# Autodesk Inventor assembly: ENSAMBLE DEL MOLDE DE INYECCION
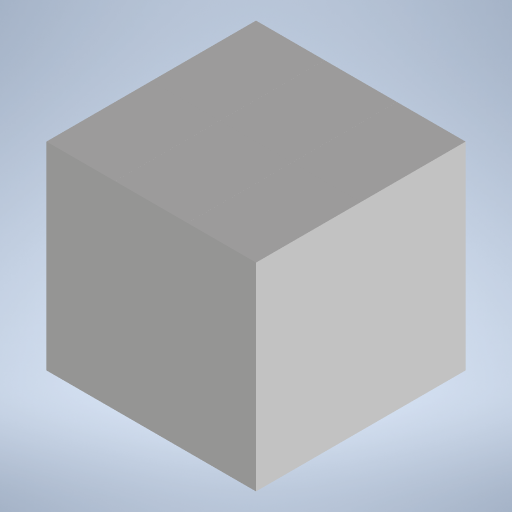
[picture p0: Inventor's stored thumbnail of the model, 512x512]
Saved by Autodesk Inventor 2024 (Build 280153000, 153)
## iProperties
Created: 2023-08-25
Part Number: ENSAMBLE DEL MOLDE DE INYECCION
Document SubType Name: Assembly
Designer: gdpg
Author: gdpg
## Documents named in this file (19)
- C:\Users\gdpg\Desktop\MANIQUI\MODELO FINAL\MOLDE\ENSAMBLE DEL MOLDE DE INYECCION.iam
- C:\Users\gdpg\Desktop\MANIQUI\MODELO FINAL\MOLDE\1.ipt
- C:\Users\gdpg\Desktop\MANIQUI\MODELO FINAL\MOLDE\2.ipt
- C:\Users\gdpg\Desktop\MANIQUI\MODELO FINAL\MOLDE\3.ipt
- C:\Users\gdpg\Desktop\MANIQUI\MODELO FINAL\MOLDE\4.ipt
- C:\Users\gdpg\Desktop\MANIQUI\MODELO FINAL\MOLDE\11.ipt
- C:\Users\gdpg\Desktop\MANIQUI\MODELO FINAL\MOLDE\12.ipt
- C:\Users\gdpg\Desktop\MANIQUI\MODELO FINAL\MOLDE\7.ipt
- C:\Users\gdpg\Desktop\MANIQUI\MODELO FINAL\MOLDE\8.ipt
- C:\Users\gdpg\Desktop\MANIQUI\MODELO FINAL\MOLDE\5.ipt
- C:\Users\gdpg\Desktop\MANIQUI\MODELO FINAL\MOLDE\6.ipt
- C:\Users\gdpg\Desktop\MANIQUI\MODELO FINAL\MOLDE\9.ipt
- C:\Users\gdpg\Desktop\MANIQUI\MODELO FINAL\MOLDE\10.ipt
- C:\Users\gdpg\Desktop\MANIQUI\MODELO FINAL\MOLDE\13.ipt
- C:\Users\gdpg\Desktop\MANIQUI\MODELO FINAL\MOLDE\14.ipt
- C:\Users\gdpg\Desktop\MANIQUI\MODELO FINAL\MOLDE\15.ipt
- C:\Users\gdpg\Desktop\MANIQUI\MODELO FINAL\MOLDE\16.ipt
- C:\Users\gdpg\Desktop\MANIQUI\MODELO FINAL\MOLDE\17.ipt
- C:\Users\gdpg\Desktop\MANIQUI\MODELO FINAL\MOLDE\18.ipt
## Components (18 placed, 18 different names)
1. 1:1 — Nivelación:1, Coincidencia:1, Coincidencia:2, Coincidencia:15, Coincidencia:16, Coincidencia:19, Coincidencia:20, Coincidencia:23, Coincidencia:28, Coincidencia:32
2. 2:1 — Nivelación:1, Coincidencia:5, Coincidencia:6, Coincidencia:26, Coincidencia:29
3. 3:1 — Coincidencia:19, Coincidencia:20, Coincidencia:21, Coincidencia:22, Coincidencia:31
4. 4:1 — Coincidencia:21, Coincidencia:22, Coincidencia:33
5. 5:1 — Coincidencia:13, Coincidencia:14, Coincidencia:24
6. 6:1 — Coincidencia:11, Coincidencia:12
7. 7:1 — Coincidencia:1, Coincidencia:2, Coincidencia:3, Coincidencia:4, Coincidencia:7, Coincidencia:8, Coincidencia:13, Coincidencia:14
8. 8:1 — Coincidencia:3, Coincidencia:4, Coincidencia:5, Coincidencia:6, Coincidencia:11, Coincidencia:12
9. 9:1 — Coincidencia:15, Coincidencia:16, Coincidencia:17, Coincidencia:18
10. 10:1 — Coincidencia:17, Coincidencia:18
11. 11:1 — Coincidencia:7, Coincidencia:8, Coincidencia:9, Coincidencia:10, Coincidencia:27
12. 12:1 — Coincidencia:9, Coincidencia:10, Coincidencia:30
13. 13:1 — Coincidencia:23, Coincidencia:24, Coincidencia:25
14. 14:1 — Coincidencia:25, Coincidencia:26
15. 15:1 — Coincidencia:27, Coincidencia:28
16. 16:1 — Coincidencia:29, Coincidencia:30
17. 17:1 — Coincidencia:31, Coincidencia:32, Coincidencia:34
18. 18:1 — Coincidencia:33, Coincidencia:34
## Relationships (35: Mate 34, Flush 1)
- Nivelación:1 [Flush]: 1:1 ↔ 2:1
- Coincidencia:1 [Mate]: 1:1 ↔ 7:1
- Coincidencia:2 [Mate]: 1:1 ↔ 7:1
- Coincidencia:3 [Mate]: 7:1 ↔ 8:1
- Coincidencia:4 [Mate]: 7:1 ↔ 8:1
- Coincidencia:5 [Mate]: 2:1 ↔ 8:1
- Coincidencia:6 [Mate]: 2:1 ↔ 8:1
- Coincidencia:7 [Mate]: 7:1 ↔ 11:1
- Coincidencia:8 [Mate]: 7:1 ↔ 11:1
- Coincidencia:9 [Mate]: 11:1 ↔ 12:1
- Coincidencia:10 [Mate]: 11:1 ↔ 12:1
- Coincidencia:11 [Mate]: 6:1 ↔ 8:1
- Coincidencia:12 [Mate]: 6:1 ↔ 8:1
- Coincidencia:13 [Mate]: 5:1 ↔ 7:1
- Coincidencia:14 [Mate]: 5:1 ↔ 7:1
- Coincidencia:15 [Mate]: 1:1 ↔ 9:1
- Coincidencia:16 [Mate]: 1:1 ↔ 9:1
- Coincidencia:17 [Mate]: 9:1 ↔ 10:1
- Coincidencia:18 [Mate]: 9:1 ↔ 10:1
- Coincidencia:19 [Mate]: 1:1 ↔ 3:1
- Coincidencia:20 [Mate]: 1:1 ↔ 3:1
- Coincidencia:21 [Mate]: 3:1 ↔ 4:1
- Coincidencia:22 [Mate]: 3:1 ↔ 4:1
- Coincidencia:23 [Mate]: 1:1 ↔ 13:1
- Coincidencia:24 [Mate]: 5:1 ↔ 13:1
- Coincidencia:25 [Mate]: 13:1 ↔ 14:1
- Coincidencia:26 [Mate]: 2:1 ↔ 14:1
- Coincidencia:27 [Mate]: 11:1 ↔ 15:1
- Coincidencia:28 [Mate]: 1:1 ↔ 15:1
- Coincidencia:29 [Mate]: 2:1 ↔ 16:1
- Coincidencia:30 [Mate]: 12:1 ↔ 16:1
- Coincidencia:31 [Mate]: 3:1 ↔ 17:1
- Coincidencia:32 [Mate]: 1:1 ↔ 17:1
- Coincidencia:33 [Mate]: 4:1 ↔ 18:1
- Coincidencia:34 [Mate]: 17:1 ↔ 18:1
